# Autodesk Inventor assembly: Electronics
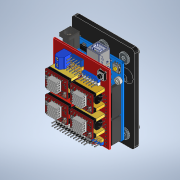
[picture p0: Inventor's stored thumbnail of the model, 180x180]
Saved by Autodesk Inventor 2022 (Build 260153000, 153)
## iProperties
Created: 2022-03-15
Part Number: Electronics
Document SubType Name: Assembly
Designer: JK
Author: JK
## Documents named in this file (5)
- C:\Users\JK\Documents\Inventor\ScaraNema\SCARA-3DP\Parts\Electronics\Electronics.iam
- C:\Users\JK\Documents\Inventor\ScaraNema\SCARA-3DP\Parts\Electronics\Electronics base.ipt
- C:\Users\JK\Documents\Inventor\ScaraNema\SCARA-3DP\Parts\Electronics\Arduino UNO and Shield\Arduino_CNC_Assembly.iam
- C:\Users\JK\Documents\Inventor\ScaraNema\SCARA-3DP\Parts\Electronics\M3x10.ipt
- C:\Users\JK\Documents\Inventor\ScaraNema\SCARA-3DP\Parts\Electronics\M5x12 flathead.ipt
## Components (9 placed, 4 different names)
1. Electronics base:1 — Nivelación:1, Nivelación:2, Coincidencia:1, Coincidencia:8, Coincidencia:9, Coincidencia:10, Coincidencia:11
2. Arduino_CNC_Assembly:1 [sub-assembly] — Nivelación:1, Nivelación:2, Coincidencia:1, Coincidencia:2, Coincidencia:3, Coincidencia:4, Coincidencia:5, Coincidencia:6, Coincidencia:7
3. M3x10:1 — Coincidencia:4, Nivelación:4
4. M3x10:2 — Coincidencia:3, Coincidencia:7, Nivelación:3
5. M3x10:3 — Coincidencia:5, Coincidencia:6
6. M3x10:4 — Coincidencia:2, Nivelación:3, Nivelación:4
7. M5x12 flathead:1 — Coincidencia:8, Nivelación:6, Coincidencia:11
8. M5x12 flathead:2 — Coincidencia:10, Nivelación:5
9. M5x12 flathead:3 — Coincidencia:9, Nivelación:5, Nivelación:6
## Relationships (17: Mate 11, Flush 6)
- Nivelación:1 [Flush] (5 mm): Electronics base:1 ↔ Arduino_CNC_Assembly:1
- Nivelación:2 [Flush] (5 mm): Electronics base:1 ↔ Arduino_CNC_Assembly:1
- Coincidencia:1 [Mate]: Electronics base:1 ↔ Arduino_CNC_Assembly:1
- Coincidencia:2 [Mate]: Arduino_CNC_Assembly:1 ↔ M3x10:4
- Coincidencia:3 [Mate]: Arduino_CNC_Assembly:1 ↔ M3x10:2
- Coincidencia:4 [Mate]: Arduino_CNC_Assembly:1 ↔ M3x10:1
- Coincidencia:5 [Mate]: Arduino_CNC_Assembly:1 ↔ M3x10:3
- Coincidencia:6 [Mate]: Arduino_CNC_Assembly:1 ↔ M3x10:3
- Coincidencia:7 [Mate]: Arduino_CNC_Assembly:1 ↔ M3x10:2
- Nivelación:3 [Flush]: M3x10:2 ↔ M3x10:4
- Nivelación:4 [Flush]: M3x10:1 ↔ M3x10:4
- Coincidencia:8 [Mate]: Electronics base:1 ↔ M5x12 flathead:1
- Coincidencia:9 [Mate]: Electronics base:1 ↔ M5x12 flathead:3
- Coincidencia:10 [Mate]: Electronics base:1 ↔ M5x12 flathead:2
- Nivelación:5 [Flush]: M5x12 flathead:2 ↔ M5x12 flathead:3
- Nivelación:6 [Flush]: M5x12 flathead:1 ↔ M5x12 flathead:3
- Coincidencia:11 [Mate]: Electronics base:1 ↔ M5x12 flathead:1
